# Autodesk Inventor assembly: Pont arriere
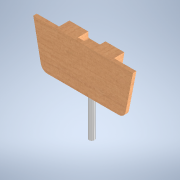
[picture p0: Inventor's stored thumbnail of the model, 180x180]
Saved by Autodesk Inventor 2021 (Build 250183000, 183)
## iProperties
Created: 2021-01-15
Part Number: Pont arriere
Document SubType Name: Assembly
Designer: dimercur
Author: dimercur
## Documents named in this file (3)
- C:\Users\dimercur\Travail\Projets Git\voilier\meca\Equerres porte carte\Pont arriere.iam
- C:\Users\dimercur\Travail\Projets Git\voilier\meca\Equerres porte carte\Pont arriere.ipt
- C:\Users\dimercur\Travail\Projets Git\voilier\meca\Equerres porte carte\Tube alu.ipt
## Components (2 placed, 2 different names)
1. Pont arriere:1 — Placage:1, Placage:2
2. Tube alu:1 — Placage:1, Placage:2
## Relationships (2: Mate 2)
- Placage:1 [Mate]: Pont arriere:1 ↔ Tube alu:1
- Placage:2 [Mate]: Pont arriere:1 ↔ Tube alu:1
